# Autodesk Inventor assembly: full_shaft_small
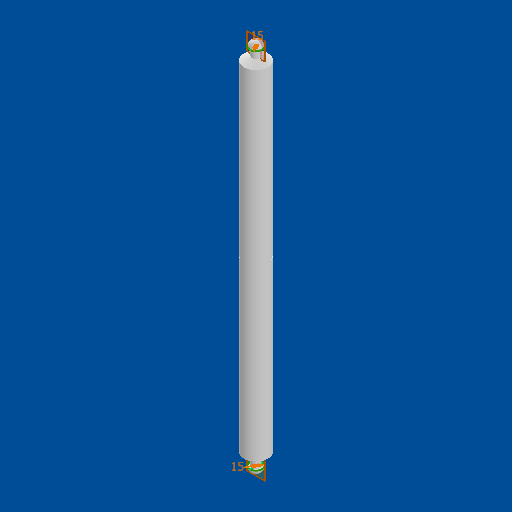
[picture p0: Inventor's stored thumbnail of the model, 512x512]
Saved by Autodesk Inventor 2026.2 (Build 302298000, 298)
## iProperties
Created: 2026-02-18
Part Number: full_shaft_small
Document SubType Name: Assembly
Designer: Thoma
Author: Thoma
## Documents named in this file (2)
- C:\Users\Thoma\OneDrive\Desktop\dir\telescope_cover\telescope\version_3\full_shaft_small.iam
- C:\Users\Thoma\OneDrive\Desktop\dir\telescope_cover\telescope\version_3\Shafts_small.ipt
## Components (2 placed, 1 different names)
1. Shafts_small:1 — Mate:1, Mate:2
2. Shafts_small:2 — Mate:1, Mate:2
## Relationships (2: Mate 2)
- Mate:1: Shafts_small:1 ↔ Shafts_small:2
- Mate:2: Shafts_small:1 ↔ Shafts_small:2
